# Autodesk Inventor assembly: AM14U4 Long Half
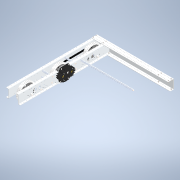
[picture p0: Inventor's stored thumbnail of the model, 180x180]
Saved by Autodesk Inventor 2020 (Build 240168000, 168)
## iProperties
Created: 2020-01-25
Part Number: AM14U4 Long Half
Document SubType Name: Assembly
Designer: 1cikaychapman
Author: 1cikaychapman
Revision Number: ANY
## Documents named in this file (10)
- C:\Users\autum\Google Drive\Iron Riders 4180 (Roosevelt Robotics)\2019-2020\Build_Design\Robot 2020 (1)\Chassis\AM14U4 Long Half.iam
- C:\Users\autum\Google Drive\Iron Riders 4180 (Roosevelt Robotics)\2019-2020\Build_Design\Robot 2020 (1)\Chassis\AM14U4 Long Frame Half.iam
- C:\Users\autum\Google Drive\Iron Riders 4180 (Roosevelt Robotics)\2019-2020\Build_Design\Robot 2020 (1)\Chassis\6 HiGrip with bearings, pulleys and spacers.iam
- C:\Users\autum\Google Drive\Iron Riders 4180 (Roosevelt Robotics)\2019-2020\Build_Design\Robot 2020 (1)\Chassis\am-2598_107 2016 KOP Toughbox Mini.iam
- C:\Users\autum\Google Drive\Iron Riders 4180 (Roosevelt Robotics)\2019-2020\Build_Design\Robot 2020 (1)\Chassis\FR8ZZ Hex Bearing.ipt
- C:\Users\autum\Google Drive\Iron Riders 4180 (Roosevelt Robotics)\2019-2020\Build_Design\Robot 2020 (1)\Chassis\6 HiGrip with hub and double pulley.iam
- C:\Users\autum\Google Drive\Iron Riders 4180 (Roosevelt Robotics)\2019-2020\Build_Design\Robot 2020 (1)\Chassis\375-16 x 4.25 Hex Bolt_HFBOLT 0.375-16x2.5x1-C.ipt
- C:\Users\autum\Google Drive\Iron Riders 4180 (Roosevelt Robotics)\2019-2020\Build_Design\Robot 2020 (1)\Chassis\375-16 Lock Nut_91831A127.ipt
- C:\Users\autum\Google Drive\Iron Riders 4180 (Roosevelt Robotics)\2019-2020\Build_Design\Robot 2020 (1)\Chassis\800-5M-15 v2.ipt
- C:\Users\autum\Google Drive\Iron Riders 4180 (Roosevelt Robotics)\2019-2020\Build_Design\Robot 2020 (1)\Chassis\NEO.ipt
## Components (14 placed, 13 different names)
1. AM14U4 Long Frame Half_3 [sub-assembly]
2. 6 HiGrip with bearings, pulleys and spacers_4 [sub-assembly]
3. 6 HiGrip with bearings, pulleys and spacers_5 [sub-assembly]
4. am-2598_107 2016 KOP Toughbox Mini_6 [sub-assembly] — Insert:1, Insert:2
5. FR8ZZ Hex Bearing_7
6. 6 HiGrip with hub and double pulley_8 [sub-assembly]
7. 375-16 x 4.25 Hex Bolt_HFBOLT 0.375-16x2.5x1-C_9
8. 375-16 x 4.25 Hex Bolt_HFBOLT 0.375-16x2.5x1-C_10
9. 375-16 Lock Nut_91831A127_11
10. 375-16 Lock Nut_91831A127_12
11. 800-5M-15 v2_13
12. 800-5M-15 v2_14
13. NEO:1 — Insert:2
14. NEO:2 — Insert:1
## Relationships (2: Insert 2)
- Insert:1: am-2598_107 2016 KOP Toughbox Mini_6 ↔ NEO:2
- Insert:2: am-2598_107 2016 KOP Toughbox Mini_6 ↔ NEO:1
